# Autodesk Inventor assembly: Ensamblaje1
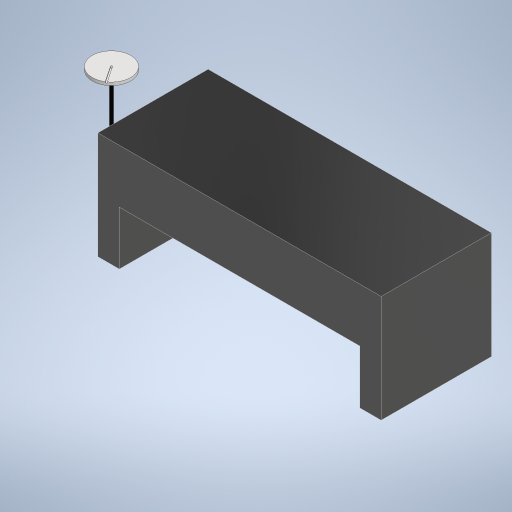
[picture p0: Inventor's stored thumbnail of the model, 512x512]
Saved by Autodesk Inventor 2024 (Build 280153000, 153)
## iProperties
Created: 2023-11-25
Part Number: Ensamblaje1
Document SubType Name: Assembly
Designer: sergi
Author: sergi
## Documents named in this file (6)
- C:\Users\sergi\OneDrive\Escritorio\proyectos\LamparaSalon\Ensamblaje1.iam
- C:\Users\sergi\OneDrive\Escritorio\proyectos\LamparaSalon\Barra.ipt
- C:\Users\sergi\OneDrive\Escritorio\proyectos\LamparaSalon\Processed_Acople E27.ipt
- C:\Users\sergi\OneDrive\Escritorio\proyectos\LamparaSalon\Casquillo.ipt
- C:\Users\sergi\OneDrive\Escritorio\proyectos\LamparaSalon\Pie.ipt
- C:\Users\sergi\OneDrive\Escritorio\proyectos\LamparaSalon\sofa.ipt
## Components (5 placed, 5 different names)
1. Barra:1 — Coincidencia:1, Nivelación:1, Coincidencia:2, Nivelación:2, Coincidencia:4, Coincidencia:5
2. Processed_Acople E27:1 — Coincidencia:1, Nivelación:1, Coincidencia:3
3. Casquillo:1 — Coincidencia:2, Coincidencia:3
4. Pie:1 — Nivelación:2, Coincidencia:4, Coincidencia:5, Nivelación:3
5. sofa:1 — Nivelación:3
## Relationships (8: Mate 5, Flush 3)
- Coincidencia:1 [Mate]: Barra:1 ↔ Processed_Acople E27:1
- Nivelación:1 [Flush]: Barra:1 ↔ Processed_Acople E27:1
- Coincidencia:2 [Mate]: Barra:1 ↔ Casquillo:1
- Coincidencia:3 [Mate]: Processed_Acople E27:1 ↔ Casquillo:1
- Nivelación:2 [Flush]: Barra:1 ↔ Pie:1
- Coincidencia:4 [Mate]: Barra:1 ↔ Pie:1
- Coincidencia:5 [Mate]: Barra:1 ↔ Pie:1
- Nivelación:3 [Flush]: Pie:1 ↔ sofa:1
